# Autodesk Inventor assembly: DeCruster Main
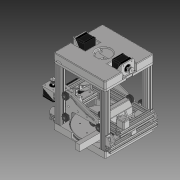
[picture p0: Inventor's stored thumbnail of the model, 180x180]
Saved by Autodesk Inventor 2020 (Build 240168000, 168)
## iProperties
Created: 2020-10-19
Part Number: DeCruster Main
Document SubType Name: Assembly
Designer: DDeGo
Author: DDeGo
## Documents named in this file (16)
- C:\Users\DDeGo\Documents\Drew\Projects\De-Cruster\cad\DeCruster Main.iam
- C:\Users\DDeGo\Documents\Drew\Projects\De-Cruster\cad\Base.ipt
- C:\Users\DDeGo\Documents\Drew\Projects\De-Cruster\cad\Turntable.ipt
- C:\Users\DDeGo\Documents\Drew\Projects\De-Cruster\cad\2020 Extrusion 200mm.ipt
- C:\Users\DDeGo\Documents\Drew\Projects\De-Cruster\cad\Carrier.iam
- C:\Users\DDeGo\Documents\Drew\Projects\De-Cruster\cad\Knifey Bit.iam
- C:\Users\DDeGo\Documents\Drew\Projects\De-Cruster\cad\Topper.ipt
- C:\Users\DDeGo\Documents\Drew\Projects\De-Cruster\cad\2020 Extrusion 135mm.ipt
- C:\Users\DDeGo\Documents\Drew\Projects\De-Cruster\cad\Nema 17.ipt
- C:\Users\DDeGo\Documents\Drew\Projects\De-Cruster\cad\ZIdler.ipt
- C:\Users\DDeGo\Documents\Drew\Projects\De-Cruster\cad\GT2 Idler Pulley.ipt
- C:\Users\DDeGo\Documents\Drew\Projects\De-Cruster\cad\127 x 146.05 x 12.7mm Printable Bearing Part 1.ipt
- C:\Users\DDeGo\Documents\Drew\Projects\De-Cruster\cad\127 x 146.05 x 12.7mm Printable Bearing Part 2.ipt
- C:\Users\DDeGo\Documents\Drew\Projects\De-Cruster\cad\MotorBracket2.ipt
- C:\Users\DDeGo\Documents\Drew\Projects\De-Cruster\cad\HBLFSNF5_b.ipt
- C:\Users\DDeGo\Documents\Drew\Projects\De-Cruster\cad\Lid.ipt
## Components (29 placed, 15 different names)
1. Base:1 — Mate:1, Mate:3, Mate:8, Angle:3, Mate:15, Mate:16, Mate:29, Mate:30, Mate:31, Mate:32, Mate:33, Mate:34, Mate:45
2. Turntable:1 — Mate:1, Mate:43, Mate:44, Flush:16
3. 2020 Extrusion 200mm:1 — Flush:6, Mate:12, Mate:13, Mate:29, Mate:32, Flush:10, Mate:55, Flush:18
4. 2020 Extrusion 200mm:2 — Mate:17, Flush:9, Mate:30, Mate:34, Flush:10, Mate:56, Flush:17
5. 2020 Extrusion 200mm:3 — Mate:11, Mate:31, Mate:33, Flush:11, Mate:54, Flush:20, Tangent:4, Tangent:5
6. 2020 Extrusion 200mm:4 — Mate:3, Mate:8, Angle:3, Flush:8, Mate:14, Flush:11, Mate:53, Flush:19
7. Carrier:1 [sub-assembly] — Flush:6, Flush:7, Tangent:2, Tangent:3, Tangent:4, Tangent:5
8. Knifey Bit:1 [sub-assembly] — Flush:7, Tangent:2, Tangent:3
9. Topper:1 — Mate:11, Mate:12, Mate:13, Mate:18, Mate:19, Mate:20, Mate:21, Mate:22, Mate:23, Mate:59, Flush:21, Flush:22
10. 2020 Extrusion 135mm:1 — Mate:16, Mate:17, Flush:9, Mate:25, Mate:27, Mate:57, Mate:58
11. 2020 Extrusion 135mm:2 — Flush:8, Mate:14, Mate:15, Mate:26, Mate:28, Mate:46, Mate:47, Flush:15, Mate:51, Mate:52
12. Nema 17:1 — Mate:18, Mate:22, Mate:23, Mate:35
13. Nema 17:2 — Mate:19, Mate:20, Mate:21, Mate:36
14. Nema 17:3 — Mate:39, Mate:48, Mate:49, Mate:50
15. ZIdler:1 — Mate:26, Mate:28, Mate:37, Mate:40
16. ZIdler:2 — Mate:25, Mate:27, Mate:38, Mate:41
17. GT2 Idler Pulley:1 — Mate:35, Flush:13
18. GT2 Idler Pulley:2 — Mate:36, Flush:12
19. GT2 Idler Pulley:3 — Mate:37, Mate:40, Flush:12
20. GT2 Idler Pulley:4 — Mate:38, Mate:41, Flush:13
21. GT2 Idler Pulley:5 — Mate:39, Flush:16
22. 127 x 146.05 x 12.7mm Printable Bearing Part 1:1 — Mate:42, Flush:14, Mate:43, Mate:44
23. 127 x 146.05 x 12.7mm Printable Bearing Part 2:2 — Mate:42, Flush:14, Mate:45
24. MotorBracket2:1 — Mate:46, Mate:47, Mate:48, Mate:49, Mate:50, Flush:15
25. HBLFSNF5_b:7 — Mate:56, Mate:57, Flush:17
26. HBLFSNF5_b:8 — Mate:55, Mate:58, Flush:18
27. HBLFSNF5_b:9 — Mate:51, Mate:53, Flush:19
28. HBLFSNF5_b:10 — Mate:52, Mate:54, Flush:20
29. Lid:1 — Mate:59, Flush:21, Flush:22
## Relationships (73: Mate 51, Flush 17, Tangent 4, Angle 1)
- Mate:1: Base:1 ↔ Turntable:1
- Mate:3: Base:1 ↔ 2020 Extrusion 200mm:4
- Mate:8: Base:1 ↔ 2020 Extrusion 200mm:4
- Angle:3 (0 deg): Base:1 ↔ 2020 Extrusion 200mm:4
- Flush:6 (5 mm): 2020 Extrusion 200mm:1 ↔ Carrier:1
- Flush:7 (-5 mm): Carrier:1 ↔ Knifey Bit:1
- Tangent:2: Carrier:1 ↔ Knifey Bit:1
- Tangent:3: Carrier:1 ↔ Knifey Bit:1
- Mate:11: 2020 Extrusion 200mm:3 ↔ Topper:1
- Mate:12: 2020 Extrusion 200mm:1 ↔ Topper:1
- Mate:13: 2020 Extrusion 200mm:1 ↔ Topper:1
- Flush:8: 2020 Extrusion 200mm:4 ↔ 2020 Extrusion 135mm:2
- Mate:14: 2020 Extrusion 200mm:4 ↔ 2020 Extrusion 135mm:2
- Mate:15: Base:1 ↔ 2020 Extrusion 135mm:2
- Mate:16: Base:1 ↔ 2020 Extrusion 135mm:1
- Mate:17: 2020 Extrusion 200mm:2 ↔ 2020 Extrusion 135mm:1
- Flush:9: 2020 Extrusion 200mm:2 ↔ 2020 Extrusion 135mm:1
- Mate:18: Topper:1 ↔ Nema 17:1
- Mate:19: Topper:1 ↔ Nema 17:2
- Mate:20: Topper:1 ↔ Nema 17:2
- Mate:21: Topper:1 ↔ Nema 17:2
- Mate:22: Topper:1 ↔ Nema 17:1
- Mate:23: Topper:1 ↔ Nema 17:1
- Mate:25: 2020 Extrusion 135mm:1 ↔ ZIdler:2
- Mate:26: 2020 Extrusion 135mm:2 ↔ ZIdler:1
- Mate:27: 2020 Extrusion 135mm:1 ↔ ZIdler:2
- Mate:28: 2020 Extrusion 135mm:2 ↔ ZIdler:1
- Mate:29: Base:1 ↔ 2020 Extrusion 200mm:1
- Mate:30: Base:1 ↔ 2020 Extrusion 200mm:2
- Mate:31: Base:1 ↔ 2020 Extrusion 200mm:3
- Mate:32: Base:1 ↔ 2020 Extrusion 200mm:1
- Mate:33: Base:1 ↔ 2020 Extrusion 200mm:3
- Mate:34: Base:1 ↔ 2020 Extrusion 200mm:2
- Flush:10: 2020 Extrusion 200mm:1 ↔ 2020 Extrusion 200mm:2
- Flush:11: 2020 Extrusion 200mm:3 ↔ 2020 Extrusion 200mm:4
- Mate:35: Nema 17:1 ↔ GT2 Idler Pulley:1
- Mate:36: Nema 17:2 ↔ GT2 Idler Pulley:2
- Mate:37: ZIdler:1 ↔ GT2 Idler Pulley:3
- Mate:38: ZIdler:2 ↔ GT2 Idler Pulley:4
- Mate:39: Nema 17:3 ↔ GT2 Idler Pulley:5
- Mate:40 (0.25 mm): ZIdler:1 ↔ GT2 Idler Pulley:3
- Mate:41 (0.25 mm): ZIdler:2 ↔ GT2 Idler Pulley:4
- Flush:12: GT2 Idler Pulley:2 ↔ GT2 Idler Pulley:3
- Flush:13: GT2 Idler Pulley:1 ↔ GT2 Idler Pulley:4
- Mate:42: 127 x 146.05 x 12.7mm Printable Bearing Part 1:1 ↔ 127 x 146.05 x 12.7mm Printable Bearing Part 2:2
- Flush:14: 127 x 146.05 x 12.7mm Printable Bearing Part 1:1 ↔ 127 x 146.05 x 12.7mm Printable Bearing Part 2:2
- Mate:43: Turntable:1 ↔ 127 x 146.05 x 12.7mm Printable Bearing Part 1:1
- Mate:44: Turntable:1 ↔ 127 x 146.05 x 12.7mm Printable Bearing Part 1:1
- Mate:45: Base:1 ↔ 127 x 146.05 x 12.7mm Printable Bearing Part 2:2
- Mate:46: 2020 Extrusion 135mm:2 ↔ MotorBracket2:1
- Mate:47: 2020 Extrusion 135mm:2 ↔ MotorBracket2:1
- Mate:48: Nema 17:3 ↔ MotorBracket2:1
- Mate:49: Nema 17:3 ↔ MotorBracket2:1
- Mate:50: Nema 17:3 ↔ MotorBracket2:1
- Flush:15 (30 mm): 2020 Extrusion 135mm:2 ↔ MotorBracket2:1
- Flush:16: Turntable:1 ↔ GT2 Idler Pulley:5
- Mate:51: 2020 Extrusion 135mm:2 ↔ HBLFSNF5_b:9
- Mate:52: 2020 Extrusion 135mm:2 ↔ HBLFSNF5_b:10
- Mate:53: 2020 Extrusion 200mm:4 ↔ HBLFSNF5_b:9
- Mate:54: 2020 Extrusion 200mm:3 ↔ HBLFSNF5_b:10
- Mate:55: 2020 Extrusion 200mm:1 ↔ HBLFSNF5_b:8
- Mate:56: 2020 Extrusion 200mm:2 ↔ HBLFSNF5_b:7
- Mate:57: 2020 Extrusion 135mm:1 ↔ HBLFSNF5_b:7
- Mate:58: 2020 Extrusion 135mm:1 ↔ HBLFSNF5_b:8
- Flush:17: 2020 Extrusion 200mm:2 ↔ HBLFSNF5_b:7
- Flush:18: 2020 Extrusion 200mm:1 ↔ HBLFSNF5_b:8
- Flush:19: 2020 Extrusion 200mm:4 ↔ HBLFSNF5_b:9
- Flush:20: 2020 Extrusion 200mm:3 ↔ HBLFSNF5_b:10
- Tangent:4: 2020 Extrusion 200mm:3 ↔ Carrier:1
- Tangent:5: 2020 Extrusion 200mm:3 ↔ Carrier:1
- Mate:59: Topper:1 ↔ Lid:1
- Flush:21: Topper:1 ↔ Lid:1
- Flush:22: Topper:1 ↔ Lid:1
